# Autodesk Inventor assembly: Assembly_SO-OCT_v2
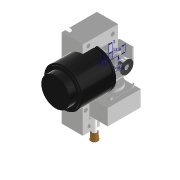
[picture p0: Inventor's stored thumbnail of the model, 180x180]
Saved by Autodesk Inventor 2022 (Build 260153000, 153)
## iProperties
Created: 2023-01-02
Part Number: Assembly_SO-OCT_v2
Document SubType Name: Assembly
Designer: diederichbenedict
Author: diederichbenedict
## Documents named in this file (18)
- C:\Users\diederichbenedict\Dropbox\Dokumente\Promotion\PROJECTS\SO-OCT\INVENTOR\Assembly_SO-OCT_v2.iam
- C:\Users\diederichbenedict\Dropbox\Dokumente\Promotion\PROJECTS\SO-OCT\INVENTOR\00_10x_Objective_ViewSolutions_bm05073332.ipt
- C:\Users\diederichbenedict\Dropbox\Dokumente\Promotion\PROJECTS\SO-OCT\INVENTOR\00_BS_KES400A_4mm.ipt
- C:\Users\diederichbenedict\Dropbox\Dokumente\Promotion\PROJECTS\SO-OCT\INVENTOR\00_VCM_M12.ipt
- C:\Users\diederichbenedict\Dropbox\Dokumente\Promotion\PROJECTS\SO-OCT\INVENTOR\00_Magnet_8x3mm.ipt
- C:\Users\diederichbenedict\Dropbox\Dokumente\Promotion\PROJECTS\SO-OCT\INVENTOR\00_F3SS25-Step.ipt
- C:\Users\diederichbenedict\Dropbox\Dokumente\Promotion\PROJECTS\SO-OCT\INVENTOR\00_F3SSN1P-Step.ipt
- C:\Users\diederichbenedict\Dropbox\Dokumente\Promotion\PROJECTS\SO-OCT\INVENTOR\01_optical_beam_path.ipt
- C:\Users\diederichbenedict\Dropbox\Dokumente\Promotion\PROJECTS\SO-OCT\INVENTOR\00_mirror_tmp.ipt
- C:\Users\diederichbenedict\Dropbox\Dokumente\Promotion\PROJECTS\SO-OCT\INVENTOR\10_SOOCT_VCM_Mount_v0.ipt
- C:\Users\diederichbenedict\Dropbox\Dokumente\Promotion\PROJECTS\SO-OCT\INVENTOR\10_SOOCT_Base_v0_MIR.ipt
- C:\Users\diederichbenedict\Dropbox\Dokumente\Promotion\PROJECTS\SO-OCT\INVENTOR\tmp_20_Cube_Insert_Kinematic_Astromedia_30x40x90_pro_magnetic_M12lens_mirrormount.ipt
- C:\Users\diederichbenedict\Dropbox\Dokumente\Promotion\PROJECTS\SO-OCT\INVENTOR\Assembly_Cube_empty_IM_v3.iam
- C:\Users\diederichbenedict\Dropbox\Dokumente\Promotion\PROJECTS\SO-OCT\INVENTOR\20_Cube_Insert_SO-OCT_Samplemount.ipt
- C:\Users\diederichbenedict\Dropbox\Dokumente\Promotion\PROJECTS\SO-OCT\INVENTOR\00_Bearing_8mm.ipt
- C:\Users\diederichbenedict\Dropbox\Dokumente\Promotion\PROJECTS\SO-OCT\INVENTOR\10_SOOCT_Base_v1.ipt
- C:\Users\diederichbenedict\Dropbox\Dokumente\Promotion\PROJECTS\SO-OCT\INVENTOR\10_SOOCT_Cube_Mount_v1.ipt
- C:\Users\diederichbenedict\Dropbox\Dokumente\Promotion\PROJECTS\SO-OCT\INVENTOR\10_SOOCT_Base_v1_MIR.ipt
## Components (22 placed, 17 different names)
1. 00_10x_Objective_ViewSolutions_bm05073332:1 — Fluchtend:1, Fluchtend:2, Fluchtend:3, Fluchtend:4, Fluchtend:5, Passend:9, Passend:16
2. 00_VCM_M12:1 — Passend:5, Passend:6, Fluchtend:5, Fluchtend:6, Fluchtend:7, Einfügen:7
3. 01_optical_beam_path:1 — Fluchtend:1, Passend:1, Passend:2, Passend:3, Passend:5, Passend:9, Passend:10, Passend:11
4. 00_mirror_tmp:1 — Fluchtend:2, Fluchtend:3, Passend:1
5. 00_mirror_tmp:2 — Fluchtend:4, Passend:2, Passend:3, Passend:6
6. 00_BS_KES400A_4mm:1 — Passend:10, Passend:11
7. 10_SOOCT_Base_v1:1 — Fluchtend:6, Passend:17, Passend:18, Einfügen:9, Fluchtend:11
8. 10_SOOCT_VCM_Mount_v0:1 — Fluchtend:7, Einfügen:6, Passend:12, Passend:14
9. 00_Magnet_8x3mm:3 — Einfügen:6
10. 00_F3SSN1P-Step:3 — Passend:13
11. 00_F3SS25-Step:3 — Passend:12, Passend:13
12. 00_F3SS25-Step:4 — Passend:14, Passend:15
13. 00_F3SSN1P-Step:4 — Passend:15
14. 10_SOOCT_Base_v0_MIR:1 — Einfügen:8, Passend:17, Passend:18, Winkel:1
15. tmp_20_Cube_Insert_Kinematic_Astromedia_30x40x90_pro_magnetic_M12lens_mirrormount:1 — Einfügen:7
16. 00_Magnet_8x3mm:4 — Einfügen:8
17. Assembly_Cube_empty_IM_v3:1 [sub-assembly] — Passend:16, Winkel:1, Fluchtend:8, Fluchtend:9, Passend:19
18. 20_Cube_Insert_SO-OCT_Samplemount:1 — Fluchtend:8, Fluchtend:9, Passend:19
19. 00_Bearing_8mm:1 — Einfügen:9, Fluchtend:10
20. 10_SOOCT_Cube_Mount_v1:1 — Fluchtend:10, Fluchtend:11
21. 10_SOOCT_Base_v1_MIR:1 — Einfügen:10
22. 00_Bearing_8mm:2 — Einfügen:10
## Relationships (33: Mate 16, Flush 11, Insert 5, Angle 1)
- Fluchtend:1 [Flush]: 00_10x_Objective_ViewSolutions_bm05073332:1 ↔ 01_optical_beam_path:1
- Fluchtend:2 [Flush]: 00_10x_Objective_ViewSolutions_bm05073332:1 ↔ 00_mirror_tmp:1
- Fluchtend:3 [Flush]: 00_10x_Objective_ViewSolutions_bm05073332:1 ↔ 00_mirror_tmp:1
- Passend:1 [Mate]: 01_optical_beam_path:1 ↔ 00_mirror_tmp:1
- Fluchtend:4 [Flush]: 00_10x_Objective_ViewSolutions_bm05073332:1 ↔ 00_mirror_tmp:2
- Passend:2 [Mate]: 01_optical_beam_path:1 ↔ 00_mirror_tmp:2
- Passend:3 [Mate]: 01_optical_beam_path:1 ↔ 00_mirror_tmp:2
- Passend:5 [Mate] (2 mm): 00_VCM_M12:1 ↔ 01_optical_beam_path:1
- Passend:6 [Mate] (6 mm): 00_VCM_M12:1 ↔ 00_mirror_tmp:2
- Fluchtend:5 [Flush]: 00_10x_Objective_ViewSolutions_bm05073332:1 ↔ 00_VCM_M12:1
- Passend:9 [Mate]: 00_10x_Objective_ViewSolutions_bm05073332:1 ↔ 01_optical_beam_path:1
- Passend:10 [Mate]: 01_optical_beam_path:1 ↔ 00_BS_KES400A_4mm:1
- Passend:11 [Mate]: 01_optical_beam_path:1 ↔ 00_BS_KES400A_4mm:1
- Fluchtend:6 [Flush] (8 mm): 00_VCM_M12:1 ↔ 10_SOOCT_Base_v1:1
- Fluchtend:7 [Flush]: 00_VCM_M12:1 ↔ 10_SOOCT_VCM_Mount_v0:1
- Einfügen:6 [Insert]: 10_SOOCT_VCM_Mount_v0:1 ↔ 00_Magnet_8x3mm:3
- Passend:12 [Mate]: 10_SOOCT_VCM_Mount_v0:1 ↔ 00_F3SS25-Step:3
- Passend:13 [Mate]: 00_F3SSN1P-Step:3 ↔ 00_F3SS25-Step:3
- Passend:14 [Mate]: 10_SOOCT_VCM_Mount_v0:1 ↔ 00_F3SS25-Step:4
- Passend:15 [Mate]: 00_F3SS25-Step:4 ↔ 00_F3SSN1P-Step:4
- Einfügen:7 [Insert] (0.1 mm): 00_VCM_M12:1 ↔ tmp_20_Cube_Insert_Kinematic_Astromedia_30x40x90_pro_magnetic_M12lens_mirrormount:1
- Einfügen:8 [Insert]: 10_SOOCT_Base_v0_MIR:1 ↔ 00_Magnet_8x3mm:4
- Passend:16 [Mate]: 00_10x_Objective_ViewSolutions_bm05073332:1 ↔ Assembly_Cube_empty_IM_v3:1
- Passend:17 [Mate]: 10_SOOCT_Base_v1:1 ↔ 10_SOOCT_Base_v0_MIR:1
- Passend:18 [Mate]: 10_SOOCT_Base_v1:1 ↔ 10_SOOCT_Base_v0_MIR:1
- Winkel:1 [Angle] (180 deg): 10_SOOCT_Base_v0_MIR:1 ↔ Assembly_Cube_empty_IM_v3:1
- Fluchtend:8 [Flush]: Assembly_Cube_empty_IM_v3:1 ↔ 20_Cube_Insert_SO-OCT_Samplemount:1
- Fluchtend:9 [Flush]: Assembly_Cube_empty_IM_v3:1 ↔ 20_Cube_Insert_SO-OCT_Samplemount:1
- Passend:19 [Mate]: Assembly_Cube_empty_IM_v3:1 ↔ 20_Cube_Insert_SO-OCT_Samplemount:1
- Einfügen:9 [Insert]: 10_SOOCT_Base_v1:1 ↔ 00_Bearing_8mm:1
- Fluchtend:10 [Flush]: 00_Bearing_8mm:1 ↔ 10_SOOCT_Cube_Mount_v1:1
- Fluchtend:11 [Flush]: 10_SOOCT_Base_v1:1 ↔ 10_SOOCT_Cube_Mount_v1:1
- Einfügen:10 [Insert]: 10_SOOCT_Base_v1_MIR:1 ↔ 00_Bearing_8mm:2
